# Autodesk Inventor assembly: Arm
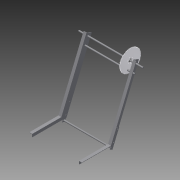
[picture p0: Inventor's stored thumbnail of the model, 180x180]
Saved by Autodesk Inventor 2013 (Build 170138000, 138)
## iProperties
Created: 2014-01-20
Part Number: Arm
Document SubType Name: Assembly
Designer: RobertB
Author: RobertB
## Documents named in this file (8)
- E:\Robotics\FRC\2014\CAD\Robot\Catapult\Arm.iam
- E:\Robotics\FRC\2014\CAD\Robot\Catapult\CatapultArm-Left.ipt
- E:\Robotics\FRC\2014\CAD\Robot\Catapult\CatapultArm-Right.ipt
- E:\Robotics\FRC\2014\CAD\Robot\Catapult\CatapultAxle.ipt
- E:\Robotics\FRC\2014\CAD\Robot\Catapult\CatapultAxleSupport.ipt
- E:\Robotics\FRC\2014\CAD\Robot\Catapult\CatapultSprocket.ipt
- E:\Robotics\FRC\2014\CAD\Robot\Catapult\BarHolder.ipt
- E:\Robotics\FRC\2014\CAD\Robot\Catapult\CrossBrace.ipt
## Components (8 placed, 7 different names)
1. CatapultArm-Left:1 — Flush:1, Flush:2, Mate:1, Mate:2, Mate:3, Mate:6, Mate:7, Mate:8, Flush:3, Flush:4
2. CatapultArm-Right:1 — Flush:1, Flush:2, Mate:1, Mate:4, Mate:5, Mate:9, Mate:10, Mate:11
3. CatapultAxle:1 — Mate:4, Flush:3
4. CatapultAxleSupport:1 — Mate:5, Mate:14, Flush:4
5. CatapultSprocket:1 — Mate:2, Mate:3, Mate:14
6. BarHolder:1 — Mate:6, Mate:7, Mate:8
7. BarHolder:2 — Mate:9, Mate:10, Mate:11, Mate:12, Mate:13
8. CrossBrace:1 — Mate:12, Mate:13
## Relationships (18: Mate 14, Flush 4)
- Flush:1: CatapultArm-Left:1 ↔ CatapultArm-Right:1
- Flush:2: CatapultArm-Left:1 ↔ CatapultArm-Right:1
- Mate:1 (406.4 mm): CatapultArm-Left:1 ↔ CatapultArm-Right:1
- Mate:2: CatapultArm-Left:1 ↔ CatapultSprocket:1
- Mate:3 (38.1 mm): CatapultArm-Left:1 ↔ CatapultSprocket:1
- Mate:4: CatapultArm-Right:1 ↔ CatapultAxle:1
- Mate:5: CatapultArm-Right:1 ↔ CatapultAxleSupport:1
- Mate:6: CatapultArm-Left:1 ↔ BarHolder:1
- Mate:7: CatapultArm-Left:1 ↔ BarHolder:1
- Mate:8: CatapultArm-Left:1 ↔ BarHolder:1
- Mate:9: CatapultArm-Right:1 ↔ BarHolder:2
- Mate:10: CatapultArm-Right:1 ↔ BarHolder:2
- Mate:11: CatapultArm-Right:1 ↔ BarHolder:2
- Mate:12: BarHolder:2 ↔ CrossBrace:1
- Mate:13: BarHolder:2 ↔ CrossBrace:1
- Mate:14: CatapultAxleSupport:1 ↔ CatapultSprocket:1
- Flush:3 (69.85 mm): CatapultArm-Left:1 ↔ CatapultAxle:1
- Flush:4 (22.225 mm): CatapultArm-Left:1 ↔ CatapultAxleSupport:1
